# Autodesk Inventor assembly: WingAssembly
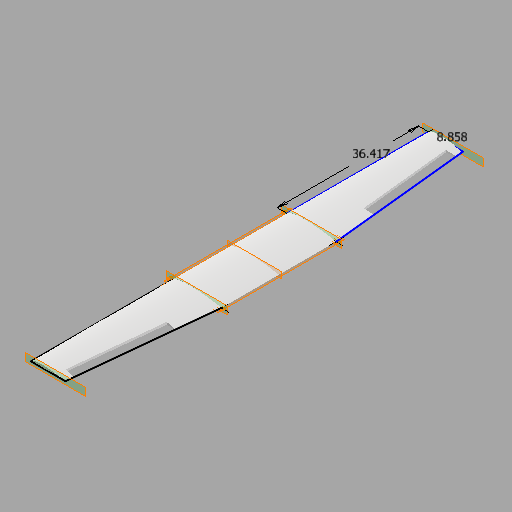
[picture p0: Inventor's stored thumbnail of the model, 512x512]
Saved by Autodesk Inventor 2025 (Build 290162000, 162)
## iProperties
Created: 2025-06-04
Part Number: WingAssembly
Document SubType Name: Assembly
Designer: Cupri
Author: Cupri
## Documents named in this file (4)
- C:\Users\Cupri\OneDrive - University of South Carolina\Lab projects\UAV\SWIFT-UAV\System_development\v0.1\SubAssemblies\WingAssembly\WingAssembly.iam
- C:\Users\Cupri\OneDrive - University of South Carolina\Lab projects\UAV\SWIFT-UAV\System_development\v0.1\Parts\MiddleWing.ipt
- C:\Users\Cupri\OneDrive - University of South Carolina\Lab projects\UAV\SWIFT-UAV\System_development\v0.1\Parts\OuterWingRight.ipt
- C:\Users\Cupri\OneDrive - University of South Carolina\Lab projects\UAV\SWIFT-UAV\System_development\v0.1\Parts\OuterWingLeft.ipt
## Components (3 placed, 3 different names)
1. MiddleWing:1 — Mate:1, Mate:2
2. OuterWingRight:1 — Mate:1, Mate:2
3. OuterWingLeft:1
## Relationships (2: Mate 2)
- Mate:1: MiddleWing:1 ↔ OuterWingRight:1
- Mate:2: MiddleWing:1 ↔ OuterWingRight:1
